# Autodesk Inventor assembly: Synchronous Belts Transmission
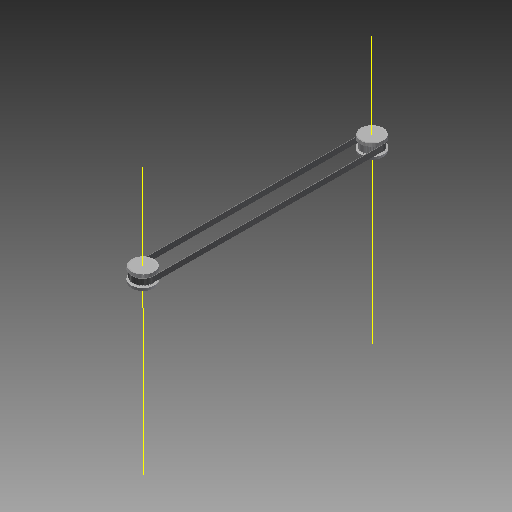
[picture p0: Inventor's stored thumbnail of the model, 512x512]
Saved by Autodesk Inventor 2017 (Build 210142000, 142)
## iProperties
Created: 2017-11-17
Part Number: Synchronous Belts Transmission
Document SubType Name: Assembly
Designer: Biscuit
ClientObjectVersion: 1
Author: Biscuit
## Documents named in this file (4)
- C:\Users\Biscuit\Google Drive\ENSEIRB\EIRBOT\COUPE 2018\Cubes\assemblage\Design Accelerator\Synchronous Belts Transmission1.iam
- C:\Users\Biscuit\Google Drive\ENSEIRB\EIRBOT\COUPE 2018\Cubes\assemblage\Design Accelerator\Synchronous Belt1.ipt
- C:\Users\Biscuit\Google Drive\ENSEIRB\EIRBOT\COUPE 2018\Cubes\assemblage\Design Accelerator\Synchronous Pulley11.ipt
- C:\Users\Biscuit\Google Drive\ENSEIRB\EIRBOT\COUPE 2018\Cubes\assemblage\Design Accelerator\Synchronous Pulley21.ipt
## Components (3 placed, 3 different names)
1. Synchronous Belt:1 — Flush:1, Mate:1, Mate:2, Flush:2, Mate:3, Mate:4
2. Synchronous Pulley1:1 — Flush:1, Mate:1, Mate:2, Rotation:1
3. Synchronous Pulley2:1 — Flush:2, Mate:3, Rotation:1, Mate:4
## Relationships (7: Mate 4, Flush 2, RelateRotation 1)
- Flush:1: Synchronous Belt:1 ↔ Synchronous Pulley1:1
- Mate:1: Synchronous Belt:1 ↔ Synchronous Pulley1:1
- Mate:2: Synchronous Belt:1 ↔ Synchronous Pulley1:1
- Flush:2: Synchronous Belt:1 ↔ Synchronous Pulley2:1
- Mate:3: Synchronous Belt:1 ↔ Synchronous Pulley2:1
- Rotation:1 [RelateRotation] (1 ul): Synchronous Pulley1:1 ↔ Synchronous Pulley2:1
- Mate:4: Synchronous Belt:1 ↔ Synchronous Pulley2:1
